# Autodesk Inventor assembly: gears
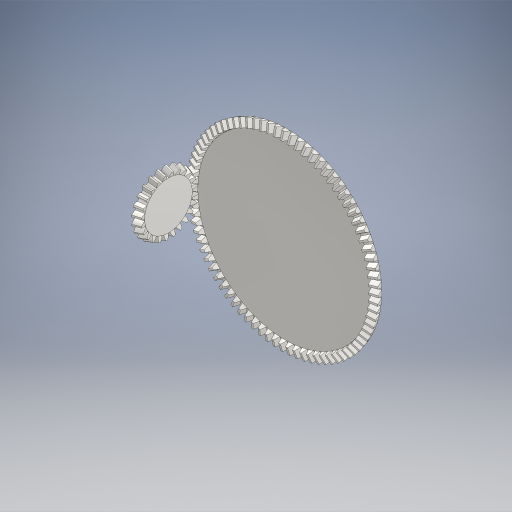
[picture p0: Inventor's stored thumbnail of the model, 512x512]
Saved by Autodesk Inventor 2024 (Build 280153000, 153)
## iProperties
Created: 2024-04-10
Part Number: gears
Document SubType Name: Assembly
Designer: Alex
Author: Alex
## Documents named in this file (3)
- C:\Shared\alex-bartella-schoolwork\4z03\final\gears.iam
- C:\Shared\alex-bartella-schoolwork\4z03\final\large bevel gear.ipt
- C:\Shared\alex-bartella-schoolwork\4z03\final\small bevel gear.ipt
## Components (2 placed, 2 different names)
1. Bevel Gear2:1 — Flush:1, Mate:2, Rotation:1
2. Bevel Gear1:1 — Mate:1, Rotation:1, Mate:3
## Relationships (5: Mate 3, Flush 1, RelateRotation 1)
- Flush:1: Bevel Gear2:1
- Mate:1: Bevel Gear1:1
- Mate:2: Bevel Gear2:1
- Rotation:1 [RelateRotation] (0.3 ul): Bevel Gear2:1 ↔ Bevel Gear1:1
- Mate:3 (-120 mm): Bevel Gear1:1
